# Autodesk Inventor assembly: Assembly1
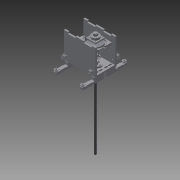
[picture p0: Inventor's stored thumbnail of the model, 180x180]
Saved by Autodesk Inventor 2015 (Build 190159000, 159)
## iProperties
Created: 2017-03-07
Part Number: Assembly1
Document SubType Name: Assembly
Designer: Ernest
Author: Ernest
## Documents named in this file (25)
- C:\Users\1esh9\Documents\Capstone-Project\doc\CAD\EndEffectorBase2\Assembly1.iam
- C:\Users\1esh9\Documents\Capstone-Project\doc\CAD\EndEffectorBase2\ThreadBar90.ipt
- C:\Users\1esh9\Documents\Capstone-Project\doc\CAD\Stepper Motor\NEMA-17\NEMA 17.iam
- C:\Users\1esh9\Documents\Capstone-Project\doc\CAD\Gears\Spur Gears1.iam
- C:\Users\1esh9\Documents\Capstone-Project\doc\CAD\Sensors\LinesensorHolderBottom.ipt
- C:\Users\1esh9\Documents\Capstone-Project\doc\CAD\Sensors\LinesensorHolderTop.ipt
- C:\Users\1esh9\Documents\Capstone-Project\doc\CAD\Sensors\LinesensorHolderWasher.ipt
- C:\Users\1esh9\Documents\Capstone-Project\doc\CAD\EndEffectorBase2\BigPositionDisk.ipt
- C:\Users\1esh9\Documents\Capstone-Project\doc\CAD\EndEffectorBase2\SmallPositionDisk.ipt
- C:\Users\1esh9\Documents\Capstone-Project\doc\CAD\LowLevel_Rev3\EE_base\EE_base_assembly.iam
- C:\Users\1esh9\Documents\Capstone-Project\doc\CAD\EndEffectorBase2\BallBearing.ipt
- C:\Users\1esh9\Documents\Capstone-Project\doc\CAD\EndEffectorBase2\BallBearingCenterer.ipt
- C:\Users\1esh9\Documents\Capstone-Project\doc\CAD\EndEffectorBase2\9mmRodNut.ipt
- C:\Users\1esh9\Documents\Capstone-Project\doc\CAD\EndEffectorBase2\BallBearingHolderTop.ipt
- C:\Users\1esh9\Documents\Capstone-Project\doc\CAD\EndEffectorBase2\BallBearingHolderBottom.ipt
- C:\Users\1esh9\Documents\Capstone-Project\doc\CAD\Sensors\TestMount.ipt
- C:\Users\1esh9\Documents\Capstone-Project\doc\CAD\EndEffectorBase2\MotorBracket.ipt
- C:\Users\1esh9\Documents\Capstone-Project\doc\CAD\Nuts and Bolts\SensorBolt-M3x11.ipt
- C:\Users\1esh9\Documents\Capstone-Project\doc\CAD\Sensors\LinesensorHolderBottomRound.ipt
- C:\Users\1esh9\Documents\Capstone-Project\doc\CAD\Sensors\LinesensorHolderTopRound.ipt
- C:\Users\1esh9\Documents\Capstone-Project\doc\CAD\Sensors\LinesensorHolderWasherRound.ipt
- C:\Users\1esh9\Documents\Capstone-Project\doc\CAD\Sensors\LinesensorHolderMidRound.ipt
- C:\Users\1esh9\Documents\Capstone-Project\doc\CAD\Wheels-Pulleys\Wheel.ipt
- C:\Users\1esh9\Documents\Capstone-Project\doc\CAD\Wheels-Pulleys\WheelYBottom.ipt
- C:\Users\1esh9\Documents\Capstone-Project\doc\CAD\EndEffectorBase2\BottomWheelHolder.ipt
## Components (43 placed, 24 different names)
1. ThreadBar90:1 — Mate:14, Mate:22, Mate:23, Mate:24, Mate:25, Mate:31, Mate:41, Mate:42, Mate:59, Mate:60, Mate:72, Mate:73
2. NEMA 17:1 [sub-assembly] — Mate:1, Mate:26, Mate:32, Mate:43, Mate:44, Mate:45, Mate:46, Angle:4, Mate:47, Mate:48, Mate:49, Mate:50, Mate:51, Mate:52, Mate:58
3. Spur Gears:1 [sub-assembly] — Mate:1, Mate:14, Mate:16, Mate:17, Mate:28, Mate:56
4. LinesensorHolderBottom:2 — Mate:5, Mate:6, Mate:7, Mate:43, Angle:4
5. LinesensorHolderTop:2 — Mate:2, Mate:3, Mate:4, Mate:5, Mate:7, Mate:38, Mate:39, Mate:40
6. LinesensorHolderWasher:1 — Mate:2, Mate:3, Mate:4, Mate:6
7. LinesensorHolderWasher:2 — Flush:5, Mate:59, Mate:60, Flush:7, Mate:64, Flush:8, Mate:80
8. BigPositionDisk:1 — Mate:31, Flush:5
9. SmallPositionDisk:1 — Mate:32, Mate:38, Mate:39, Mate:40
10. EE_base_assembly:1 [sub-assembly] — Flush:1, Mate:33, Mate:57, Mate:73, Angle:5, Angle:6, Mate:74, Mate:75, Mate:76, Mate:77, Flush:14, Flush:16, Mate:85, Flush:17, Mate:87, Mate:88, Mate:89, Angle:7, Flush:25
11. BallBearing:1 — Mate:16, Mate:20, Flush:3, Mate:27
12. BallBearing:2 — Mate:17, Flush:1, Mate:21, Flush:2, Mate:26
13. BallBearingCenterer:1 — Mate:20, Flush:3
14. BallBearingCenterer:2 — Mate:21, Flush:2
15. 9mmRodNut:1 — Mate:24
16. 9mmRodNut:2 — Mate:25
17. 9mmRodNut:3 — Mate:22
18. 9mmRodNut:4 — Mate:23
19. BallBearingHolderTop:1 — Mate:27, Mate:28, Mate:33
20. BallBearingHolderBottom:1 — Mate:56, Mate:57, Mate:58, Angle:5
21. 9mmRodNut:5 — Mate:41
22. 9mmRodNut:6 — Mate:42
23. TestMount:1 — Mate:44, Mate:45, Mate:46
24. MotorBracket:1 — Mate:48, Mate:50, Mate:52, Mate:55
25. MotorBracket:2 — Mate:47, Mate:49, Mate:51, Mate:53, Mate:54
26. SensorBolt-M3x11:1 — Flush:4, Mate:55
27. SensorBolt-M3x11:2 — Flush:4, Mate:53, Mate:54
28. LinesensorHolderBottomRound:1 — Mate:65, Flush:9, Mate:69, Mate:71, Mate:80
29. LinesensorHolderTopRound:1 — Mate:66, Mate:68, Flush:10, Mate:69
30. LinesensorHolderWasherRound:1 — Flush:7, Mate:64, Flush:8, Mate:65, Mate:66, Mate:68, Flush:9, Flush:10
31. LinesensorHolderMidRound:1 — Mate:71, Mate:72, Angle:6
32. Wheel:1 — Mate:75, Flush:12, Mate:81
33. Wheel:2 — Mate:74, Flush:12
34. Wheel:3 — Mate:77, Flush:13
35. Wheel:4 — Mate:76, Flush:13, Mate:81, Flush:16
36. WheelYBottom:1 — Flush:15, Mate:90, Flush:23
37. WheelYBottom:2 — Flush:14, Flush:15, Mate:86, Flush:24
38. BottomWheelHolder:3 — Mate:85, Flush:17, Mate:86, Flush:18, Flush:21
39. BottomWheelHolder:4 — Mate:87, Flush:18, Flush:22, Mate:90, Flush:25
40. BottomWheelHolder:5 — Mate:88, Flush:19, Flush:20, Flush:22, Mate:92
41. BottomWheelHolder:6 — Mate:89, Flush:19, Angle:7, Flush:20, Flush:21, Mate:91
42. WheelYBottom:3 — Mate:92, Flush:23
43. WheelYBottom:4 — Mate:91, Flush:24
## Relationships (94: Mate 67, Flush 23, Angle 4)
- Mate:1: NEMA 17:1 ↔ Spur Gears:1
- Mate:2: LinesensorHolderTop:2 ↔ LinesensorHolderWasher:1
- Mate:3: LinesensorHolderTop:2 ↔ LinesensorHolderWasher:1
- Mate:4: LinesensorHolderTop:2 ↔ LinesensorHolderWasher:1
- Mate:5: LinesensorHolderBottom:2 ↔ LinesensorHolderTop:2
- Mate:6: LinesensorHolderBottom:2 ↔ LinesensorHolderWasher:1
- Mate:7: LinesensorHolderBottom:2 ↔ LinesensorHolderTop:2
- Mate:14: ThreadBar90:1 ↔ Spur Gears:1
- Mate:16: Spur Gears:1 ↔ BallBearing:1
- Mate:17: Spur Gears:1 ↔ BallBearing:2
- Flush:1: EE_base_assembly:1 ↔ BallBearing:2
- Mate:20: BallBearing:1 ↔ BallBearingCenterer:1
- Mate:21: BallBearing:2 ↔ BallBearingCenterer:2
- Flush:2 (0.4 mm): BallBearing:2 ↔ BallBearingCenterer:2
- Flush:3 (0.4 mm): BallBearing:1 ↔ BallBearingCenterer:1
- Mate:22: ThreadBar90:1 ↔ 9mmRodNut:3
- Mate:23: ThreadBar90:1 ↔ 9mmRodNut:4
- Mate:24: ThreadBar90:1 ↔ 9mmRodNut:1
- Mate:25: ThreadBar90:1 ↔ 9mmRodNut:2
- Mate:26 (5 mm): NEMA 17:1 ↔ BallBearing:2
- Mate:27: BallBearing:1 ↔ BallBearingHolderTop:1
- Mate:28: Spur Gears:1 ↔ BallBearingHolderTop:1
- Mate:31: ThreadBar90:1 ↔ BigPositionDisk:1
- Mate:32: NEMA 17:1 ↔ SmallPositionDisk:1
- Mate:33: EE_base_assembly:1 ↔ BallBearingHolderTop:1
- Mate:38 (0.2 mm): LinesensorHolderTop:2 ↔ SmallPositionDisk:1
- Mate:39 (26.387 mm): LinesensorHolderTop:2 ↔ SmallPositionDisk:1
- Mate:40 (26.387 mm): LinesensorHolderTop:2 ↔ SmallPositionDisk:1
- Mate:41: ThreadBar90:1 ↔ 9mmRodNut:5
- Mate:42: ThreadBar90:1 ↔ 9mmRodNut:6
- Mate:43 (3 mm): NEMA 17:1 ↔ LinesensorHolderBottom:2
- Mate:44: NEMA 17:1 ↔ TestMount:1
- Mate:45: NEMA 17:1 ↔ TestMount:1
- Mate:46: NEMA 17:1 ↔ TestMount:1
- Angle:4 (0 deg): NEMA 17:1 ↔ LinesensorHolderBottom:2
- Mate:47: NEMA 17:1 ↔ MotorBracket:2
- Mate:48: NEMA 17:1 ↔ MotorBracket:1
- Mate:49: NEMA 17:1 ↔ MotorBracket:2
- Mate:50: NEMA 17:1 ↔ MotorBracket:1
- Mate:51: NEMA 17:1 ↔ MotorBracket:2
- Mate:52: NEMA 17:1 ↔ MotorBracket:1
- Flush:4: SensorBolt-M3x11:1 ↔ SensorBolt-M3x11:2
- Mate:53: MotorBracket:2 ↔ SensorBolt-M3x11:2
- Mate:54: MotorBracket:2 ↔ SensorBolt-M3x11:2
- Mate:55: MotorBracket:1 ↔ SensorBolt-M3x11:1
- Mate:56: Spur Gears:1 ↔ BallBearingHolderBottom:1
- Mate:57: EE_base_assembly:1 ↔ BallBearingHolderBottom:1
- Mate:58: NEMA 17:1 ↔ BallBearingHolderBottom:1
- Flush:5 (-0.2 mm): LinesensorHolderWasher:2 ↔ BigPositionDisk:1
- Mate:59 (26.387 mm): ThreadBar90:1 ↔ LinesensorHolderWasher:2
- Mate:60 (26.387 mm): ThreadBar90:1 ↔ LinesensorHolderWasher:2
- Flush:7: LinesensorHolderWasher:2 ↔ LinesensorHolderWasherRound:1
- Mate:64 (3.2 mm): LinesensorHolderWasher:2 ↔ LinesensorHolderWasherRound:1
- Flush:8: LinesensorHolderWasher:2 ↔ LinesensorHolderWasherRound:1
- Mate:65: LinesensorHolderBottomRound:1 ↔ LinesensorHolderWasherRound:1
- Mate:66: LinesensorHolderTopRound:1 ↔ LinesensorHolderWasherRound:1
- Mate:68: LinesensorHolderTopRound:1 ↔ LinesensorHolderWasherRound:1
- Flush:9: LinesensorHolderBottomRound:1 ↔ LinesensorHolderWasherRound:1
- Flush:10: LinesensorHolderTopRound:1 ↔ LinesensorHolderWasherRound:1
- Mate:69: LinesensorHolderBottomRound:1 ↔ LinesensorHolderTopRound:1
- Mate:71: LinesensorHolderBottomRound:1 ↔ LinesensorHolderMidRound:1
- Mate:72: ThreadBar90:1 ↔ LinesensorHolderMidRound:1
- Mate:73: ThreadBar90:1 ↔ EE_base_assembly:1
- Angle:5 (0 deg): EE_base_assembly:1 ↔ BallBearingHolderBottom:1
- Angle:6 (0 deg): EE_base_assembly:1 ↔ LinesensorHolderMidRound:1
- Mate:74: EE_base_assembly:1 ↔ Wheel:2
- Mate:75: EE_base_assembly:1 ↔ Wheel:1
- Mate:76: EE_base_assembly:1 ↔ Wheel:4
- Mate:77: EE_base_assembly:1 ↔ Wheel:3
- Flush:12: Wheel:1 ↔ Wheel:2
- Flush:13: Wheel:3 ↔ Wheel:4
- Mate:80: LinesensorHolderWasher:2 ↔ LinesensorHolderBottomRound:1
- Flush:14 (13.375 mm): EE_base_assembly:1 ↔ WheelYBottom:2
- Flush:15: WheelYBottom:1 ↔ WheelYBottom:2
- Mate:81 (-97 mm): Wheel:1 ↔ Wheel:4
- Flush:16 (8.375 mm): EE_base_assembly:1 ↔ Wheel:4
- Mate:85: EE_base_assembly:1 ↔ BottomWheelHolder:3
- Flush:17: EE_base_assembly:1 ↔ BottomWheelHolder:3
- Mate:86: WheelYBottom:2 ↔ BottomWheelHolder:3
- Mate:87: EE_base_assembly:1 ↔ BottomWheelHolder:4
- Mate:88: EE_base_assembly:1 ↔ BottomWheelHolder:5
- Mate:89: EE_base_assembly:1 ↔ BottomWheelHolder:6
- Flush:18: BottomWheelHolder:3 ↔ BottomWheelHolder:4
- Flush:19: BottomWheelHolder:5 ↔ BottomWheelHolder:6
- Angle:7 (0 deg): EE_base_assembly:1 ↔ BottomWheelHolder:6
- Flush:20: BottomWheelHolder:5 ↔ BottomWheelHolder:6
- Flush:21: BottomWheelHolder:3 ↔ BottomWheelHolder:6
- Flush:22: BottomWheelHolder:4 ↔ BottomWheelHolder:5
- Mate:90: WheelYBottom:1 ↔ BottomWheelHolder:4
- Mate:91: BottomWheelHolder:6 ↔ WheelYBottom:4
- Mate:92: BottomWheelHolder:5 ↔ WheelYBottom:3
- Flush:23: WheelYBottom:1 ↔ WheelYBottom:3
- Flush:24: WheelYBottom:2 ↔ WheelYBottom:4
- Flush:25: EE_base_assembly:1 ↔ BottomWheelHolder:4
